# Autodesk Inventor assembly: ASY MSC 300 Cone tube
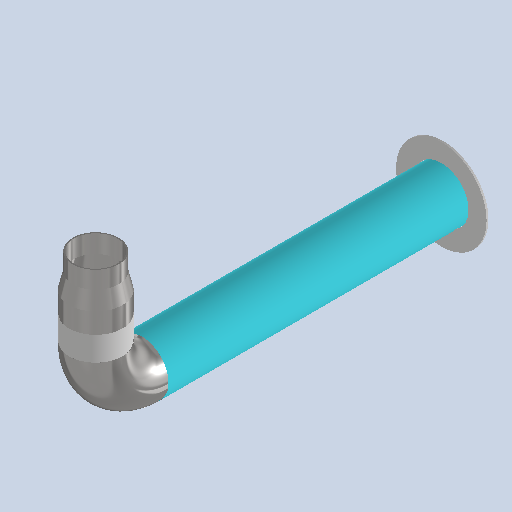
[picture p0: Inventor's stored thumbnail of the model, 512x512]
Saved by Autodesk Inventor 2025 (Build 290162010, 162A)
## iProperties
Created: 2024-08-28
Part Number: ASY MSC 300 Cone tube
Document SubType Name: Assembly
Designer: admin
Author: admin
## Documents named in this file (6)
- C:\Users\admin\YandexDisk-badmisterfox\домашниий пк\Inventor\Manturovo\Manturovo_Se-clar\ASY MSC 300 Cone tube.iam
- C:\Users\admin\YandexDisk-badmisterfox\домашниий пк\Inventor\Manturovo\Manturovo_Se-clar\ракета\МОО 064 ракета труба.ipt
- C:\Users\admin\YandexDisk-badmisterfox\домашниий пк\Inventor\Manturovo\Manturovo_Se-clar\ракета\МОО 069 ракета труба 9.ipt
- C:\Users\admin\YandexDisk-badmisterfox\домашниий пк\Inventor\Manturovo\Manturovo_Se-clar\MSC 0392 flange 2.ipt
- C:\Users\admin\YandexDisk-badmisterfox\домашниий пк\Inventor\Manturovo\Manturovo_Se-clar\Content Center Files\en-US\JIS B 2312 90 (3)\JIS B 2312 90 Deg Short Elbow Stainless Steel 80A x Sch 5S.ipt
- C:\Users\admin\YandexDisk-badmisterfox\домашниий пк\Inventor\Manturovo\Manturovo_Se-clar\Content Center Files\en-US\JIS B 2312 (1)\JIS B 2312 Concentric Reducer Stainless Steel 80A x 65A x Sch5S.ipt
## Components (5 placed, 5 different names)
1. МОО 064 ракета труба.ipt:1
2. МОО 069 ракета труба 9:1
3. MSC 0392 flange 2:1
4. JIS B 2312 90 Deg Short Elbow Stainless Steel 80A x Sch 5S:1
5. JIS B 2312 Concentric Reducer Stainless Steel 80A x 65A x Sch5S:1
## Relationships (4: WeldJoint 3, RevoluteJoint 1)
- [WeldJoint]: МОО 064 ракета труба.ipt:1 ↔ MSC 0392 flange 2:1
- [WeldJoint]: МОО 069 ракета труба 9:1 ↔ JIS B 2312 90 Deg Short Elbow Stainless Steel 80A x Sch 5S:1
- [WeldJoint]: МОО 064 ракета труба.ipt:1 ↔ JIS B 2312 90 Deg Short Elbow Stainless Steel 80A x Sch 5S:1
- [RevoluteJoint]: МОО 069 ракета труба 9:1 ↔ JIS B 2312 Concentric Reducer Stainless Steel 80A x 65A x Sch5S:1
